# Autodesk Inventor assembly: Stowed CubSat Assembly
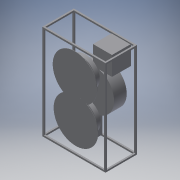
[picture p0: Inventor's stored thumbnail of the model, 180x180]
Saved by Autodesk Inventor 2016 (Build 200138000, 138)
## iProperties
Created: 2015-12-21
Part Number: Stowed CubSat Assembly
Document SubType Name: Assembly
Designer: jonathan
Author: jonathan
## Documents named in this file (6)
- C:\Users\jonathan\Dropbox\Satellite\CAD\Stowed CubSat Assembly.iam
- C:\Users\jonathan\Dropbox\Satellite\CAD\CubeSat Frame.ipt
- C:\Users\jonathan\Dropbox\Satellite\CAD\Spinning Platform.ipt
- C:\Users\jonathan\Dropbox\Satellite\CAD\Motor Assembly.iam
- C:\Users\jonathan\Dropbox\Satellite\CAD\Large Flywheel.ipt
- C:\Users\jonathan\Dropbox\Satellite\CAD\Small Flywheel Appx.ipt
## Components (8 placed, 5 different names)
1. CubeSat Frame:1 — Mate:3, Flush:1, Flush:2
2. Spinning Platform:1 — Mate:2, Rotational:2, Flush:2
3. Spinning Platform:2 — Mate:1, Rotational:1, Flush:1
4. Motor Assembly:1 [sub-assembly] — Mate:1, Rotational:1
5. Motor Assembly:2 [sub-assembly] — Mate:2, Rotational:2
6. Large Flywheel:1 — Mate:3
7. Small Flywheel Appx:1
8. Small Flywheel Appx:2
## Relationships (7: Mate 3, RevoluteJoint 2, Flush 2)
- Mate:1: Spinning Platform:2 ↔ Motor Assembly:1
- Rotational:1 [RevoluteJoint]: Spinning Platform:2 ↔ Motor Assembly:1
- Mate:2: Spinning Platform:1 ↔ Motor Assembly:2
- Rotational:2 [RevoluteJoint]: Spinning Platform:1 ↔ Motor Assembly:2
- Mate:3: CubeSat Frame:1 ↔ Large Flywheel:1
- Flush:1: CubeSat Frame:1 ↔ Spinning Platform:2
- Flush:2: CubeSat Frame:1 ↔ Spinning Platform:1
